# Autodesk Inventor assembly: PCB
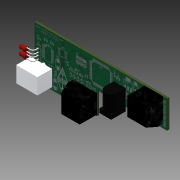
[picture p0: Inventor's stored thumbnail of the model, 180x180]
Saved by Autodesk Inventor 2014 SP1 (Build 180222100, 222)
## iProperties
Created: 2014-04-06
Part Number: PCB
Document SubType Name: Assembly
Designer: Tyler
Author: Tyler
## Documents named in this file (6)
- C:\Users\Tyler\Documents\housing\PCB\PCB.iam
- C:\Users\Tyler\Documents\housing\PCB\pcb.ipt
- C:\Users\Tyler\Documents\housing\PCB\USB_B.ipt
- C:\Users\Tyler\Documents\housing\PCB\6P6C.ipt
- C:\Users\Tyler\Documents\housing\PCB\jack.ipt
- C:\Users\Tyler\Documents\housing\PCB\led.ipt
## Components (7 placed, 5 different names)
1. pcb:1 — Flush:1, Mate:1, Flush:2, Mate:2, Flush:3, Flush:4, Mate:3, Flush:5, Flush:6, Mate:4, Flush:7, Mate:5, Mate:6, Mate:7, Mate:8, Mate:9
2. USB_B:1 — Flush:1, Mate:1, Flush:2, Tangent:1
3. 6P6C:1 — Mate:2, Flush:3, Flush:4
4. 6P6C:2 — Mate:3, Flush:5, Flush:6
5. jack:1 — Mate:4, Flush:7, Mate:5
6. led:1 — Mate:7, Mate:9, Tangent:1, Tangent:2
7. led:2 — Mate:6, Mate:8, Tangent:2
## Relationships (18: Mate 9, Flush 7, Tangent 2)
- Flush:1 (2 mm): pcb:1 ↔ USB_B:1
- Mate:1: pcb:1 ↔ USB_B:1
- Flush:2 (-3 mm): pcb:1 ↔ USB_B:1
- Mate:2: pcb:1 ↔ 6P6C:1
- Flush:3: pcb:1 ↔ 6P6C:1
- Flush:4 (1 mm): pcb:1 ↔ 6P6C:1
- Mate:3: pcb:1 ↔ 6P6C:2
- Flush:5: pcb:1 ↔ 6P6C:2
- Flush:6 (3 mm): pcb:1 ↔ 6P6C:2
- Mate:4: pcb:1 ↔ jack:1
- Flush:7 (-3 mm): pcb:1 ↔ jack:1
- Mate:5 (12.75 mm): pcb:1 ↔ jack:1
- Mate:6: pcb:1 ↔ led:2
- Mate:7: pcb:1 ↔ led:1
- Mate:8 (2 mm): pcb:1 ↔ led:2
- Mate:9 (2 mm): pcb:1 ↔ led:1
- Tangent:1 (1 mm): USB_B:1 ↔ led:1
- Tangent:2 (1.55 mm): led:1 ↔ led:2
